# Autodesk Inventor assembly: Nanoscopy-on-a-cheap_v1
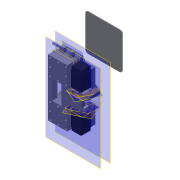
[picture p0: Inventor's stored thumbnail of the model, 180x180]
Saved by Autodesk Inventor 2019 (Build 230136000, 136)
## iProperties
Created: 2019-05-02
Part Number: Nanoscopy-on-a-cheap_v1
Document SubType Name: Assembly
Designer: diederichbenedict
Author: diederichbenedict
## Documents named in this file (12)
- C:\Users\diederichbenedict\Dropbox\Dokumente\Promotion\PROJECTS\STORMoChip\INVENTOR\Nanoscopy-on-a-cheap\Nanoscopy-on-a-cheap_v1.iam
- C:\Users\diederichbenedict\Dropbox\Dokumente\Promotion\PROJECTS\STORMoChip\INVENTOR\Nanoscopy-on-a-cheap\00_ZEISS_Axiotech_Plate.ipt
- C:\Users\diederichbenedict\Dropbox\Dokumente\Promotion\PROJECTS\STORMoChip\INVENTOR\Nanoscopy-on-a-cheap\00_XY_stage-CHUO_SEIKI_LD-647-R1.iam
- C:\Users\diederichbenedict\Dropbox\Dokumente\Promotion\PROJECTS\STORMoChip\INVENTOR\Nanoscopy-on-a-cheap\Assembly_Lasergroup_wPickup_v1.iam
- C:\Users\diederichbenedict\Dropbox\Dokumente\Promotion\PROJECTS\STORMoChip\INVENTOR\Nanoscopy-on-a-cheap\Assembly_Chipgroup.iam
- C:\Users\diederichbenedict\Dropbox\Dokumente\Promotion\PROJECTS\STORMoChip\INVENTOR\Nanoscopy-on-a-cheap\00_Microscope_Objective.ipt
- C:\Users\diederichbenedict\Dropbox\Dokumente\Promotion\PROJECTS\STORMoChip\INVENTOR\Nanoscopy-on-a-cheap\10_Adapter_Laser_XY_left.ipt
- C:\Users\diederichbenedict\Dropbox\Dokumente\Promotion\PROJECTS\STORMoChip\INVENTOR\Nanoscopy-on-a-cheap\10_Adapter_Laser_XY_right.ipt
- C:\Users\diederichbenedict\Dropbox\Dokumente\Promotion\PROJECTS\STORMoChip\INVENTOR\Nanoscopy-on-a-cheap\02_Nanoscopy_Chip.ipt
- C:\Users\diederichbenedict\Dropbox\Dokumente\Promotion\PROJECTS\STORMoChip\INVENTOR\Nanoscopy-on-a-cheap\10_Baseplate.ipt
- C:\Users\diederichbenedict\Dropbox\Dokumente\Promotion\PROJECTS\STORMoChip\INVENTOR\Nanoscopy-on-a-cheap\00_Baseplate_Axiotech.ipt
- C:\Users\diederichbenedict\Dropbox\Dokumente\Promotion\PROJECTS\STORMoChip\INVENTOR\Nanoscopy-on-a-cheap\10_Baseplate_axiotech.ipt
## Components (13 placed, 11 different names)
1. 00_ZEISS_Axiotech_Plate:1 — Mate:13
2. 00_XY_stage-CHUO_SEIKI_LD-647-R1:1 [sub-assembly] — Flush:3, Flush:6, Flush:11, Flush:12, Flush:20, Flush:22, Flush:23, Flush:25, Flush:26
3. 00_XY_stage-CHUO_SEIKI_LD-647-R1:2 [sub-assembly] — Flush:3, Mate:5, Flush:7, Insert:19, Angle:1, Flush:20, Flush:21
4. Assembly_Lasergroup_wPickup_v1:1 [sub-assembly] — Mate:3, Flush:5, Mate:5, Flush:7, Mate:15, Flush:21
5. Assembly_Lasergroup_wPickup_v1:2 [sub-assembly] — Mate:3, Flush:5, Flush:6, Mate:7, Mate:8, Mate:15, Mate:16, Mate:17, Mate:18
6. 02_Nanoscopy_Chip:1 — Mate:19
7. Assembly_Chipgroup:1 [sub-assembly] — Mate:16, Mate:17, Mate:18, Mate:19, Flush:24
8. 00_Microscope_Objective:1 — Mate:7, Mate:8, Mate:13
9. 10_Adapter_Laser_XY_left:1 — Flush:11, Flush:12
10. 10_Adapter_Laser_XY_right:1 — Insert:19, Angle:1
11. 10_Baseplate:1 — Flush:22, Flush:23, Flush:24
12. 00_Baseplate_Axiotech:1
13. 10_Baseplate_axiotech:1 — Flush:25, Flush:26
## Relationships (27: Flush 13, Mate 10, Insert 2, Angle 2)
- Flush:3: 00_XY_stage-CHUO_SEIKI_LD-647-R1:1 ↔ 00_XY_stage-CHUO_SEIKI_LD-647-R1:2
- Mate:3 (60 mm): Assembly_Lasergroup_wPickup_v1:1 ↔ Assembly_Lasergroup_wPickup_v1:2
- Flush:5: Assembly_Lasergroup_wPickup_v1:1 ↔ Assembly_Lasergroup_wPickup_v1:2
- Mate:5 (5 mm): 00_XY_stage-CHUO_SEIKI_LD-647-R1:2 ↔ Assembly_Lasergroup_wPickup_v1:1
- Flush:6: 00_XY_stage-CHUO_SEIKI_LD-647-R1:1 ↔ Assembly_Lasergroup_wPickup_v1:2
- Flush:7: 00_XY_stage-CHUO_SEIKI_LD-647-R1:2 ↔ Assembly_Lasergroup_wPickup_v1:1
- Mate:7 (30 mm): Assembly_Lasergroup_wPickup_v1:2 ↔ 00_Microscope_Objective:1
- Mate:8 (-16 mm): Assembly_Lasergroup_wPickup_v1:2 ↔ 00_Microscope_Objective:1
- Flush:11: 00_XY_stage-CHUO_SEIKI_LD-647-R1:1 ↔ 10_Adapter_Laser_XY_left:1
- Flush:12: 00_XY_stage-CHUO_SEIKI_LD-647-R1:1 ↔ 10_Adapter_Laser_XY_left:1
- Mate:13 (30 mm): 00_ZEISS_Axiotech_Plate:1 ↔ 00_Microscope_Objective:1
- Insert:19: 00_XY_stage-CHUO_SEIKI_LD-647-R1:2 ↔ 10_Adapter_Laser_XY_right:1
- Angle:1 (0 deg): 00_XY_stage-CHUO_SEIKI_LD-647-R1:2 ↔ 10_Adapter_Laser_XY_right:1
- Flush:20: 00_XY_stage-CHUO_SEIKI_LD-647-R1:1 ↔ 00_XY_stage-CHUO_SEIKI_LD-647-R1:2
- Mate:15: Assembly_Lasergroup_wPickup_v1:1 ↔ Assembly_Lasergroup_wPickup_v1:2
- [Insert] (5 mm): 02_Nanoscopy_Chip:1 ↔ 00_Microscope_Objective:1
- [Angle] (180 deg): 02_Nanoscopy_Chip:1 ↔ 10_Adapter_Laser_XY_left:1
- Mate:16 (2 mm): Assembly_Lasergroup_wPickup_v1:2 ↔ Assembly_Chipgroup:1
- Flush:21 (8 mm): 00_XY_stage-CHUO_SEIKI_LD-647-R1:2 ↔ Assembly_Lasergroup_wPickup_v1:1
- Mate:17 (3 mm): Assembly_Lasergroup_wPickup_v1:2 ↔ Assembly_Chipgroup:1
- Mate:18 (2 mm): Assembly_Lasergroup_wPickup_v1:2 ↔ Assembly_Chipgroup:1
- Mate:19 (10 mm): 02_Nanoscopy_Chip:1 ↔ Assembly_Chipgroup:1
- Flush:22: 00_XY_stage-CHUO_SEIKI_LD-647-R1:1 ↔ 10_Baseplate:1
- Flush:23: 00_XY_stage-CHUO_SEIKI_LD-647-R1:1 ↔ 10_Baseplate:1
- Flush:24: Assembly_Chipgroup:1 ↔ 10_Baseplate:1
- Flush:25: 00_XY_stage-CHUO_SEIKI_LD-647-R1:1 ↔ 10_Baseplate_axiotech:1
- Flush:26: 00_XY_stage-CHUO_SEIKI_LD-647-R1:1 ↔ 10_Baseplate_axiotech:1
